# Autodesk Inventor assembly: Assembly1
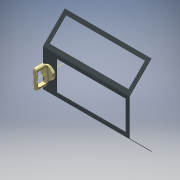
[picture p0: Inventor's stored thumbnail of the model, 180x180]
Saved by Autodesk Inventor 2016 (Build 200138000, 138)
## iProperties
Created: 2017-08-29
Part Number: Assembly1
Document SubType Name: Assembly
Designer: m207653
Author: m207653
## Documents named in this file (3)
- C:\Users\m207653\cover doors\Assembly1.iam
- C:\Users\m207653\cover doors\door.ipt
- C:\Users\m207653\cover doors\door handle.ipt
## Components (2 placed, 2 different names)
1. door:1 — Mate:1, Mate:4
2. door handle:1 — Mate:2, Rotation:1, Mate:4
## Relationships (5: Mate 4, RelateRotation 1)
- Mate:1: door:1
- Mate:2: door handle:1
- Mate:3
- Rotation:1 [RelateRotation] (10 ul): door handle:1
- Mate:4: door:1 ↔ door handle:1
